# Autodesk Inventor assembly: enc-BackPanel Oben - Assembly
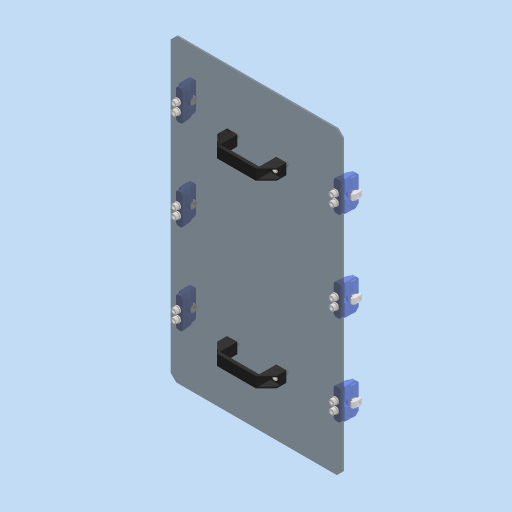
[picture p0: Inventor's stored thumbnail of the model, 512x512]
Saved by Autodesk Inventor 2023.2 (Build 272271000, 271)
## iProperties
Created: 2023-12-04
Part Number: enc-BackPanel Oben - Assembly
Document SubType Name: Assembly
Designer: Nils Bade
Author: Nils Bade
## Documents named in this file (6)
- C:\Users\nilsb\Documents\Inventor\Projektarbeit-Bade\Enclosure\enc-BackPanel Oben - Assembly.iam
- C:\Users\nilsb\Documents\Inventor\Projektarbeit-Bade\Enclosure\enc-BackPanel Unten.ipt
- C:\Users\nilsb\Documents\Inventor\Projektarbeit-Bade\Enclosure\V-Slot Door Handle v1.ipt
- C:\Users\nilsb\Documents\Inventor\Projektarbeit-Bade\Schrauben\Cap Head Screw M6x16 - DIN912.ipt
- C:\Users\nilsb\Documents\Inventor\Projektarbeit-Bade\RatRig_Standards\Hex Locking Nut - M6 v2.ipt
- C:\Users\nilsb\Documents\Inventor\Projektarbeit-Bade\Enclosure\Magnet PanelFrame 90deg connected.iam
## Components (17 placed, 5 different names)
1. enc-BackPanel Unten:1 — Passend:5, Passend:6, Passend:7, Passend:8, Passend:9, Passend:10, Passend:11, Passend:14, Passend:15, Passend:16, Passend:23, Passend:24, Passend:25, Passend:26, Passend:27, Passend:28, Passend:29, Passend:30, Passend:31, Passend:32, Passend:33, Passend:34, Passend:35, Passend:36, Passend:37, Passend:38, Passend:39, Passend:40
2. V-Slot Door Handle v1:1 — Passend:9, Passend:10, Passend:11, Passend:12, Passend:13, Passend:21, Passend:22
3. V-Slot Door Handle v1:2 — Passend:14, Passend:15, Passend:16, Passend:17, Passend:18, Passend:19, Passend:20
4. Cap Head Screw M6x16 - DIN912:1 — Passend:3, Passend:12, Passend:22
5. Cap Head Screw M6x16 - DIN912:2 — Passend:4, Passend:13, Passend:21
6. Cap Head Screw M6x16 - DIN912:3 — Passend:2, Passend:18, Passend:19
7. Cap Head Screw M6x16 - DIN912:4 — Passend:1, Passend:17, Passend:20
8. Hex Locking Nut - M6 v2:1 — Passend:3, Passend:5
9. Hex Locking Nut - M6 v2:2 — Passend:4, Passend:6
10. Hex Locking Nut - M6 v2:3 — Passend:2, Passend:8
11. Hex Locking Nut - M6 v2:4 — Passend:1, Passend:7
12. Magnet PanelFrame 90deg connected:1 [sub-assembly] — Passend:32, Passend:33, Passend:34
13. Magnet PanelFrame 90deg connected:2 [sub-assembly] — Passend:35, Passend:36, Passend:37
14. Magnet PanelFrame 90deg connected:3 [sub-assembly] — Passend:38, Passend:39, Passend:40
15. Magnet PanelFrame 90deg connected:4 [sub-assembly] — Passend:23, Passend:24, Passend:25
16. Magnet PanelFrame 90deg connected:5 [sub-assembly] — Passend:26, Passend:27, Passend:28
17. Magnet PanelFrame 90deg connected:6 [sub-assembly] — Passend:29, Passend:30, Passend:31
## Relationships (40: Mate 40)
- Passend:1 [Mate]: Cap Head Screw M6x16 - DIN912:4 ↔ Hex Locking Nut - M6 v2:4
- Passend:2 [Mate]: Cap Head Screw M6x16 - DIN912:3 ↔ Hex Locking Nut - M6 v2:3
- Passend:3 [Mate]: Cap Head Screw M6x16 - DIN912:1 ↔ Hex Locking Nut - M6 v2:1
- Passend:4 [Mate]: Cap Head Screw M6x16 - DIN912:2 ↔ Hex Locking Nut - M6 v2:2
- Passend:5 [Mate]: enc-BackPanel Unten:1 ↔ Hex Locking Nut - M6 v2:1
- Passend:6 [Mate]: enc-BackPanel Unten:1 ↔ Hex Locking Nut - M6 v2:2
- Passend:7 [Mate]: enc-BackPanel Unten:1 ↔ Hex Locking Nut - M6 v2:4
- Passend:8 [Mate]: enc-BackPanel Unten:1 ↔ Hex Locking Nut - M6 v2:3
- Passend:9 [Mate]: enc-BackPanel Unten:1 ↔ V-Slot Door Handle v1:1
- Passend:10 [Mate]: enc-BackPanel Unten:1 ↔ V-Slot Door Handle v1:1
- Passend:11 [Mate]: enc-BackPanel Unten:1 ↔ V-Slot Door Handle v1:1
- Passend:12 [Mate]: V-Slot Door Handle v1:1 ↔ Cap Head Screw M6x16 - DIN912:1
- Passend:13 [Mate]: V-Slot Door Handle v1:1 ↔ Cap Head Screw M6x16 - DIN912:2
- Passend:14 [Mate]: enc-BackPanel Unten:1 ↔ V-Slot Door Handle v1:2
- Passend:15 [Mate]: enc-BackPanel Unten:1 ↔ V-Slot Door Handle v1:2
- Passend:16 [Mate]: enc-BackPanel Unten:1 ↔ V-Slot Door Handle v1:2
- Passend:17 [Mate]: V-Slot Door Handle v1:2 ↔ Cap Head Screw M6x16 - DIN912:4
- Passend:18 [Mate]: V-Slot Door Handle v1:2 ↔ Cap Head Screw M6x16 - DIN912:3
- Passend:19 [Mate]: V-Slot Door Handle v1:2 ↔ Cap Head Screw M6x16 - DIN912:3
- Passend:20 [Mate]: V-Slot Door Handle v1:2 ↔ Cap Head Screw M6x16 - DIN912:4
- Passend:21 [Mate]: V-Slot Door Handle v1:1 ↔ Cap Head Screw M6x16 - DIN912:2
- Passend:22 [Mate]: V-Slot Door Handle v1:1 ↔ Cap Head Screw M6x16 - DIN912:1
- Passend:23 [Mate]: enc-BackPanel Unten:1 ↔ Magnet PanelFrame 90deg connected:4
- Passend:24 [Mate]: enc-BackPanel Unten:1 ↔ Magnet PanelFrame 90deg connected:4
- Passend:25 [Mate]: enc-BackPanel Unten:1 ↔ Magnet PanelFrame 90deg connected:4
- Passend:26 [Mate]: enc-BackPanel Unten:1 ↔ Magnet PanelFrame 90deg connected:5
- Passend:27 [Mate]: enc-BackPanel Unten:1 ↔ Magnet PanelFrame 90deg connected:5
- Passend:28 [Mate]: enc-BackPanel Unten:1 ↔ Magnet PanelFrame 90deg connected:5
- Passend:29 [Mate]: enc-BackPanel Unten:1 ↔ Magnet PanelFrame 90deg connected:6
- Passend:30 [Mate]: enc-BackPanel Unten:1 ↔ Magnet PanelFrame 90deg connected:6
- Passend:31 [Mate]: enc-BackPanel Unten:1 ↔ Magnet PanelFrame 90deg connected:6
- Passend:32 [Mate]: enc-BackPanel Unten:1 ↔ Magnet PanelFrame 90deg connected:1
- Passend:33 [Mate]: enc-BackPanel Unten:1 ↔ Magnet PanelFrame 90deg connected:1
- Passend:34 [Mate]: enc-BackPanel Unten:1 ↔ Magnet PanelFrame 90deg connected:1
- Passend:35 [Mate]: enc-BackPanel Unten:1 ↔ Magnet PanelFrame 90deg connected:2
- Passend:36 [Mate]: enc-BackPanel Unten:1 ↔ Magnet PanelFrame 90deg connected:2
- Passend:37 [Mate]: enc-BackPanel Unten:1 ↔ Magnet PanelFrame 90deg connected:2
- Passend:38 [Mate]: enc-BackPanel Unten:1 ↔ Magnet PanelFrame 90deg connected:3
- Passend:39 [Mate]: enc-BackPanel Unten:1 ↔ Magnet PanelFrame 90deg connected:3
- Passend:40 [Mate]: enc-BackPanel Unten:1 ↔ Magnet PanelFrame 90deg connected:3
